# Autodesk Inventor assembly: ASSY,MK4i,Swerve_Module_INV
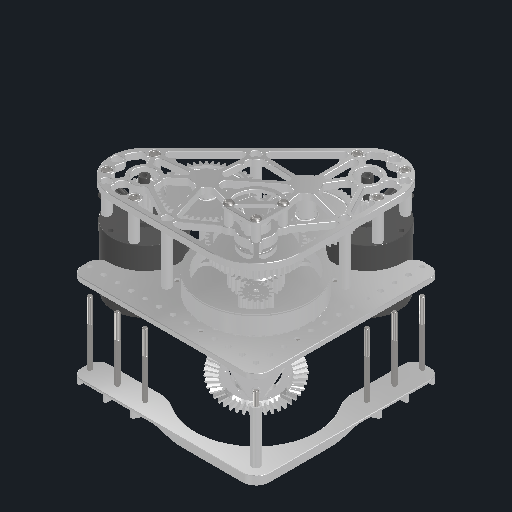
[picture p0: Inventor's stored thumbnail of the model, 512x512]
Saved by Autodesk Inventor 2025.1 (Build 291241020, 241B)
## iProperties
Created: 2025-01-13
Part Number: ASSY,MK4i,Swerve_Module_INV
Document SubType Name: Assembly
Designer: dave.simone
Mfg Approved By: John.Thibert
Mass: 2445.64 g
Surface Area: 3723.57 cm^2
Volume: 611.291 cm^3
Density: 4.00078 g/cm^3
ILogicPurgeVersion: 0.0.0.0
OnSaveVersion: 3.5.0.0
OnSaveAssembly: COREAutomationManager
ModelCat: Uncategorized
CN_MASS: 2.45
Author: dave.simone
## Documents named in this file (14)
- D:\Documents\Inventor\2025-Poseidon-Mechanical\ASSY,MK4i,Swerve_Module_INV.iam
- D:\Documents\Inventor\2025-Poseidon-Mechanical\PURCHASED_SUB,PLATE,MAIN,MK4i,Swerve.ipt
- D:\Documents\Inventor\2025-Poseidon-Mechanical\PURCHASED_SUB,PLATE,CLAMP,MK4i,Swerve.ipt
- D:\Documents\Inventor\2025-Poseidon-Mechanical\PURCHASED_SUB,PLATE,UPPER,MK4i,Swerve.ipt
- D:\Documents\Inventor\2025-Poseidon-Mechanical\PURCHASED_SUB,PLATE,ENCODER,MK4i,Swerve.ipt
- D:\Documents\Inventor\2025-Poseidon-Mechanical\PURCHASED_SUB,SPACER,SHORT,MK4i,Swerve.ipt
- D:\Documents\Inventor\2025-Poseidon-Mechanical\PURCHASED_SUB,SPACER,LONG,MK4i,Swerve.ipt
- D:\Documents\Inventor\2025-Poseidon-Mechanical\SCREW,8-32 X 2.ipt
- D:\Documents\Inventor\2025-Poseidon-Mechanical\PURCHASED_SUB,SPACER,SHORTER,MK4i,Swerve.ipt
- D:\Documents\Inventor\2025-Poseidon-Mechanical\SCREW,10-32 X 1.375.ipt
- D:\Documents\Inventor\2025-Poseidon-Mechanical\PURCHASED_SUB,GEAR_TRAIN,WHEEL,MK4i,Swerve.ipt
- D:\Documents\Inventor\2025-Poseidon-Mechanical\SCREW,BUTTON,8-32 X 0.875.ipt
- D:\Documents\Inventor\2025-Poseidon-Mechanical\SCREW,BUTTON,10-32 X 0.250.ipt
- D:\Documents\Inventor\2025-Poseidon-Mechanical\CONTROLS,MOTOR,NEO,V1.ipt
## Components (41 placed, 13 different names)
1. PURCHASED_SUB,GEAR_TRAIN,WHEEL,MK4i,Swerve.ipt:1 — Mate:20, Mate:21
2. SCREW,BUTTON,8-32 X 0.875.ipt:1 — Insert:30
3. SCREW,BUTTON,8-32 X 0.875.ipt:2 — Insert:31
4. SCREW,BUTTON,8-32 X 0.875.ipt:3 — Insert:32
5. SCREW,BUTTON,10-32 X 0.250.ipt:1 — Insert:34
6. SCREW,BUTTON,10-32 X 0.250.ipt:2 — Insert:35
7. SCREW,BUTTON,10-32 X 0.250.ipt:3 — Insert:36
8. SCREW,BUTTON,10-32 X 0.250.ipt:4 — Insert:37
9. SCREW,BUTTON,10-32 X 0.250.ipt:5 — Insert:33
10. CONTROLS,MOTOR,NEO,V1.ipt:1 — Mate:22, Mate:26, Mate:27
11. CONTROLS,MOTOR,NEO,V1.ipt:2 — Mate:23, Mate:24, Mate:25
12. PURCHASED_SUB,PLATE,CLAMP,MK4i,Swerve.ipt:1 — Mate:28, Flush:1, Flush:2, Mate:30
13. PURCHASED_SUB,SPACER,LONG,MK4i,Swerve.ipt:4 — Mate:29, Mate:30
14. SCREW,8-32 X 2.ipt:1
15. SCREW,8-32 X 2.ipt:2
16. SCREW,8-32 X 2.ipt:3
17. SCREW,8-32 X 2.ipt:4
18. SCREW,8-32 X 2.ipt:5
19. SCREW,8-32 X 2.ipt:6
20. SCREW,8-32 X 2.ipt:7 — Mate:29
21. PURCHASED_SUB,PLATE,MAIN,MK4i,Swerve.ipt:1 — Mate:6, Mate:7, Mate:8, Mate:9, Mate:20, Mate:21, Insert:33, Insert:34, Insert:35, Insert:36, Insert:37, Mate:28, Flush:1, Flush:2
22. PURCHASED_SUB,PLATE,UPPER,MK4i,Swerve.ipt:1 — Insert:4, Insert:5, Insert:6, Insert:7, Insert:8, Insert:9, Insert:10, Insert:11, Insert:12, Insert:20, Insert:21, Insert:22, Insert:24, Insert:25, Insert:26, Insert:27, Insert:28, Insert:29, Mate:22, Mate:23
23. PURCHASED_SUB,SPACER,SHORTER,MK4i,Swerve.ipt:1 — Insert:20, Mate:11
24. PURCHASED_SUB,SPACER,SHORTER,MK4i,Swerve.ipt:2 — Insert:21, Mate:12
25. PURCHASED_SUB,SPACER,SHORTER,MK4i,Swerve.ipt:3 — Insert:22, Mate:13
26. PURCHASED_SUB,PLATE,ENCODER,MK4i,Swerve.ipt:1 — Mate:11, Mate:12, Mate:13, Insert:30, Insert:31, Insert:32
27. PURCHASED_SUB,SPACER,LONG,MK4i,Swerve.ipt:1 — Insert:4, Mate:6, Mate:7
28. PURCHASED_SUB,SPACER,LONG,MK4i,Swerve.ipt:2 — Insert:5, Mate:8
29. PURCHASED_SUB,SPACER,LONG,MK4i,Swerve.ipt:3 — Insert:6, Mate:9
30. PURCHASED_SUB,SPACER,SHORT,MK4i,Swerve.ipt:1 — Insert:8
31. PURCHASED_SUB,SPACER,SHORT,MK4i,Swerve.ipt:2 — Insert:7
32. PURCHASED_SUB,SPACER,SHORT,MK4i,Swerve.ipt:3 — Insert:9, Mate:26, Mate:27
33. PURCHASED_SUB,SPACER,SHORT,MK4i,Swerve.ipt:4 — Insert:10, Mate:24, Mate:25
34. PURCHASED_SUB,SPACER,SHORT,MK4i,Swerve.ipt:5 — Insert:11
35. PURCHASED_SUB,SPACER,SHORT,MK4i,Swerve.ipt:6 — Insert:12
36. SCREW,10-32 X 1.375.ipt:1 — Insert:24
37. SCREW,10-32 X 1.375.ipt:2 — Insert:25
38. SCREW,10-32 X 1.375.ipt:3 — Insert:26
39. SCREW,10-32 X 1.375.ipt:4 — Insert:27
40. SCREW,10-32 X 1.375.ipt:5 — Insert:28
41. SCREW,10-32 X 1.375.ipt:6 — Insert:29
## Relationships (53: Insert 33, Mate 18, Flush 2)
- Insert:4: PURCHASED_SUB,PLATE,UPPER,MK4i,Swerve.ipt:1 ↔ PURCHASED_SUB,SPACER,LONG,MK4i,Swerve.ipt:1
- Insert:5: PURCHASED_SUB,PLATE,UPPER,MK4i,Swerve.ipt:1 ↔ PURCHASED_SUB,SPACER,LONG,MK4i,Swerve.ipt:2
- Insert:6: PURCHASED_SUB,PLATE,UPPER,MK4i,Swerve.ipt:1 ↔ PURCHASED_SUB,SPACER,LONG,MK4i,Swerve.ipt:3
- Mate:6: PURCHASED_SUB,PLATE,MAIN,MK4i,Swerve.ipt:1 ↔ PURCHASED_SUB,SPACER,LONG,MK4i,Swerve.ipt:1
- Mate:7: PURCHASED_SUB,PLATE,MAIN,MK4i,Swerve.ipt:1 ↔ PURCHASED_SUB,SPACER,LONG,MK4i,Swerve.ipt:1
- Mate:8: PURCHASED_SUB,PLATE,MAIN,MK4i,Swerve.ipt:1 ↔ PURCHASED_SUB,SPACER,LONG,MK4i,Swerve.ipt:2
- Mate:9: PURCHASED_SUB,PLATE,MAIN,MK4i,Swerve.ipt:1 ↔ PURCHASED_SUB,SPACER,LONG,MK4i,Swerve.ipt:3
- Insert:7: PURCHASED_SUB,PLATE,UPPER,MK4i,Swerve.ipt:1 ↔ PURCHASED_SUB,SPACER,SHORT,MK4i,Swerve.ipt:2
- Insert:8: PURCHASED_SUB,PLATE,UPPER,MK4i,Swerve.ipt:1 ↔ PURCHASED_SUB,SPACER,SHORT,MK4i,Swerve.ipt:1
- Insert:9: PURCHASED_SUB,PLATE,UPPER,MK4i,Swerve.ipt:1 ↔ PURCHASED_SUB,SPACER,SHORT,MK4i,Swerve.ipt:3
- Insert:10: PURCHASED_SUB,PLATE,UPPER,MK4i,Swerve.ipt:1 ↔ PURCHASED_SUB,SPACER,SHORT,MK4i,Swerve.ipt:4
- Insert:11: PURCHASED_SUB,PLATE,UPPER,MK4i,Swerve.ipt:1 ↔ PURCHASED_SUB,SPACER,SHORT,MK4i,Swerve.ipt:5
- Insert:12: PURCHASED_SUB,PLATE,UPPER,MK4i,Swerve.ipt:1 ↔ PURCHASED_SUB,SPACER,SHORT,MK4i,Swerve.ipt:6
- Insert:20: PURCHASED_SUB,PLATE,UPPER,MK4i,Swerve.ipt:1 ↔ PURCHASED_SUB,SPACER,SHORTER,MK4i,Swerve.ipt:1
- Insert:21: PURCHASED_SUB,PLATE,UPPER,MK4i,Swerve.ipt:1 ↔ PURCHASED_SUB,SPACER,SHORTER,MK4i,Swerve.ipt:2
- Insert:22: PURCHASED_SUB,PLATE,UPPER,MK4i,Swerve.ipt:1 ↔ PURCHASED_SUB,SPACER,SHORTER,MK4i,Swerve.ipt:3
- Mate:11: PURCHASED_SUB,SPACER,SHORTER,MK4i,Swerve.ipt:1 ↔ PURCHASED_SUB,PLATE,ENCODER,MK4i,Swerve.ipt:1
- Mate:12: PURCHASED_SUB,SPACER,SHORTER,MK4i,Swerve.ipt:2 ↔ PURCHASED_SUB,PLATE,ENCODER,MK4i,Swerve.ipt:1
- Mate:13: PURCHASED_SUB,SPACER,SHORTER,MK4i,Swerve.ipt:3 ↔ PURCHASED_SUB,PLATE,ENCODER,MK4i,Swerve.ipt:1
- Insert:24: PURCHASED_SUB,PLATE,UPPER,MK4i,Swerve.ipt:1 ↔ SCREW,10-32 X 1.375.ipt:1
- Insert:25: PURCHASED_SUB,PLATE,UPPER,MK4i,Swerve.ipt:1 ↔ SCREW,10-32 X 1.375.ipt:2
- Insert:26: PURCHASED_SUB,PLATE,UPPER,MK4i,Swerve.ipt:1 ↔ SCREW,10-32 X 1.375.ipt:3
- Insert:27: PURCHASED_SUB,PLATE,UPPER,MK4i,Swerve.ipt:1 ↔ SCREW,10-32 X 1.375.ipt:4
- Insert:28: PURCHASED_SUB,PLATE,UPPER,MK4i,Swerve.ipt:1 ↔ SCREW,10-32 X 1.375.ipt:5
- Insert:29: PURCHASED_SUB,PLATE,UPPER,MK4i,Swerve.ipt:1 ↔ SCREW,10-32 X 1.375.ipt:6
- Mate:20: PURCHASED_SUB,GEAR_TRAIN,WHEEL,MK4i,Swerve.ipt:1 ↔ PURCHASED_SUB,PLATE,MAIN,MK4i,Swerve.ipt:1
- Mate:21: PURCHASED_SUB,GEAR_TRAIN,WHEEL,MK4i,Swerve.ipt:1 ↔ PURCHASED_SUB,PLATE,MAIN,MK4i,Swerve.ipt:1
- Insert:30: SCREW,BUTTON,8-32 X 0.875.ipt:1 ↔ PURCHASED_SUB,PLATE,ENCODER,MK4i,Swerve.ipt:1
- Insert:31: SCREW,BUTTON,8-32 X 0.875.ipt:2 ↔ PURCHASED_SUB,PLATE,ENCODER,MK4i,Swerve.ipt:1
- Insert:32: SCREW,BUTTON,8-32 X 0.875.ipt:3 ↔ PURCHASED_SUB,PLATE,ENCODER,MK4i,Swerve.ipt:1
- Insert:33: SCREW,BUTTON,10-32 X 0.250.ipt:5 ↔ PURCHASED_SUB,PLATE,MAIN,MK4i,Swerve.ipt:1
- Insert:34: SCREW,BUTTON,10-32 X 0.250.ipt:1 ↔ PURCHASED_SUB,PLATE,MAIN,MK4i,Swerve.ipt:1
- Insert:35: SCREW,BUTTON,10-32 X 0.250.ipt:2 ↔ PURCHASED_SUB,PLATE,MAIN,MK4i,Swerve.ipt:1
- Insert:36: SCREW,BUTTON,10-32 X 0.250.ipt:3 ↔ PURCHASED_SUB,PLATE,MAIN,MK4i,Swerve.ipt:1
- Insert:37: SCREW,BUTTON,10-32 X 0.250.ipt:4 ↔ PURCHASED_SUB,PLATE,MAIN,MK4i,Swerve.ipt:1
- Mate:22: CONTROLS,MOTOR,NEO,V1.ipt:1 ↔ PURCHASED_SUB,PLATE,UPPER,MK4i,Swerve.ipt:1
- Mate:23: CONTROLS,MOTOR,NEO,V1.ipt:2 ↔ PURCHASED_SUB,PLATE,UPPER,MK4i,Swerve.ipt:1
- Mate:24: CONTROLS,MOTOR,NEO,V1.ipt:2 ↔ PURCHASED_SUB,SPACER,SHORT,MK4i,Swerve.ipt:4
- Mate:25: CONTROLS,MOTOR,NEO,V1.ipt:2 ↔ PURCHASED_SUB,SPACER,SHORT,MK4i,Swerve.ipt:4
- Mate:26: CONTROLS,MOTOR,NEO,V1.ipt:1 ↔ PURCHASED_SUB,SPACER,SHORT,MK4i,Swerve.ipt:3
- Mate:27: CONTROLS,MOTOR,NEO,V1.ipt:1 ↔ PURCHASED_SUB,SPACER,SHORT,MK4i,Swerve.ipt:3
- [Insert]: PURCHASED_SUB,PLATE,CLAMP,MK4i,Swerve.ipt:1 ↔ SCREW,8-32 X 2.ipt:1
- [Insert]: PURCHASED_SUB,PLATE,CLAMP,MK4i,Swerve.ipt:1 ↔ SCREW,8-32 X 2.ipt:2
- [Insert]: PURCHASED_SUB,PLATE,CLAMP,MK4i,Swerve.ipt:1 ↔ SCREW,8-32 X 2.ipt:3
- [Insert]: PURCHASED_SUB,PLATE,CLAMP,MK4i,Swerve.ipt:1 ↔ SCREW,8-32 X 2.ipt:4
- [Insert]: PURCHASED_SUB,PLATE,CLAMP,MK4i,Swerve.ipt:1 ↔ SCREW,8-32 X 2.ipt:5
- [Insert]: PURCHASED_SUB,PLATE,CLAMP,MK4i,Swerve.ipt:1 ↔ SCREW,8-32 X 2.ipt:6
- [Insert]: PURCHASED_SUB,PLATE,CLAMP,MK4i,Swerve.ipt:1 ↔ SCREW,8-32 X 2.ipt:7
- Mate:28 (76.2 mm): PURCHASED_SUB,PLATE,CLAMP,MK4i,Swerve.ipt:1 ↔ PURCHASED_SUB,PLATE,MAIN,MK4i,Swerve.ipt:1
- Flush:1: PURCHASED_SUB,PLATE,CLAMP,MK4i,Swerve.ipt:1 ↔ PURCHASED_SUB,PLATE,MAIN,MK4i,Swerve.ipt:1
- Flush:2: PURCHASED_SUB,PLATE,CLAMP,MK4i,Swerve.ipt:1 ↔ PURCHASED_SUB,PLATE,MAIN,MK4i,Swerve.ipt:1
- Mate:29: PURCHASED_SUB,SPACER,LONG,MK4i,Swerve.ipt:4 ↔ SCREW,8-32 X 2.ipt:7
- Mate:30: PURCHASED_SUB,PLATE,CLAMP,MK4i,Swerve.ipt:1 ↔ PURCHASED_SUB,SPACER,LONG,MK4i,Swerve.ipt:4
## Named parameters: d66_d35 = 0 mm, d67_d23 = 0 mm, d68_d24 = 0 mm, d69_d25 = 0 mm, d70_d26 = 0 mm, d71_d27 = 0 mm, d72_d28 = 0 mm
